# Autodesk Inventor assembly: robo-gardener-2
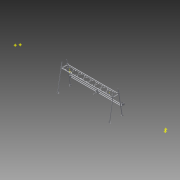
[picture p0: Inventor's stored thumbnail of the model, 180x180]
Saved by Autodesk Inventor 2013 (Build 170138000, 138)
## iProperties
Created: 2013-09-24
Part Number: robo-gardener-2
Document SubType Name: Assembly
Designer: Admin
Author: Admin
## Documents named in this file (12)
- Z:\Dropbox\projects\robo-gardener\robo-gardener-2.iam
- Z:\Dropbox\projects\robo-gardener\3d-parts\light-mount.ipt
- Z:\Dropbox\projects\robo-gardener\3d-parts\rod-long.ipt
- Z:\Dropbox\projects\robo-gardener\3d-parts\carriage-back.ipt
- Z:\Dropbox\projects\robo-gardener\3d-parts\carriage-front.ipt
- Z:\Dropbox\projects\robo-gardener\robo-gardener-2\Design Accelerator\Synchronous Belts Transmission1.iam
- Z:\Dropbox\projects\robo-gardener\3d-parts\belt-clamp.ipt
- Z:\Dropbox\projects\robo-gardener\3d-parts\motor-mount.ipt
- Z:\Dropbox\projects\robo-gardener\3d-parts\idler-mount.ipt
- Z:\Dropbox\projects\robo-gardener\3d-parts\top-connector.ipt
- Z:\Dropbox\projects\robo-gardener\3d-parts\rod-short.ipt
- Z:\Dropbox\projects\robo-gardener\3d-parts\foot.ipt
## Components (28 placed, 11 different names)
1. rod-long:1 — Insert:1, Flush:7, Insert:9, Insert:11
2. rod-long:2 — Insert:2, Mate:13, Insert:8, Insert:10
3. carriage-back:1 — Mate:1, Mate:2, Flush:9, Flush:10, Angle:1, Mate:12, Flush:13
4. carriage-front:1 — Flush:6, Mate:3, Flush:9, Flush:10, Mate:4, Flush:12, Insert:3, Insert:4, Mate:7
5. rod-long:3 — Flush:7, Flush:8, Mate:1, Mate:3, Flush:11, Mate:14, Insert:7
6. rod-long:4 — Flush:8, Mate:2, Mate:15, Insert:5, Insert:6
7. Synchronous Belts Transmission:1 [sub-assembly] — Mate:4, Mate:6, Mate:7
8. belt-clamp:1 — Flush:12, Insert:3, Insert:4
9. motor-mount:1 — Insert:5, Angle:3
10. idler-mount:1 — Insert:6, Insert:7
11. top-connector:1 — Insert:8, Insert:9, Mate:23, Mate:24
12. top-connector:2 — Insert:10, Insert:11, Mate:25, Mate:26
13. rod-short:1 — Mate:23, Insert:16
14. rod-short:2 — Mate:25, Insert:12
15. rod-short:3 — Mate:26, Insert:18
16. rod-short:4 — Mate:24, Insert:17
17. foot:1 — Insert:12, Flush:15, Flush:16, Flush:17
18. foot:2 — Insert:18, Flush:16
19. foot:3 — Insert:17, Flush:15
20. foot:4 — Insert:16, Flush:17
21. light-mount:1 — Insert:1, Insert:2, Mate:8, Flush:13
22. light-mount:2
23. light-mount:3
24. light-mount:4
25. light-mount:5
26. light-mount:6
27. light-mount:7
28. light-mount:8 — Angle:1, Mate:9
## Component patterns: (8 elements, first: light-mount:1)
## Relationships (55: Mate 25, Insert 15, Flush 12, Angle 3)
- Insert:1 (-30 mm): rod-long:1 ↔ light-mount:1
- Insert:2 (-30 mm): rod-long:2 ↔ light-mount:1
- Flush:6 (3.048 mm): carriage-front:1
- Flush:7: rod-long:1 ↔ rod-long:3
- Flush:8: rod-long:3 ↔ rod-long:4
- Mate:1: carriage-back:1 ↔ rod-long:3
- Mate:2: carriage-back:1 ↔ rod-long:4
- Mate:3: carriage-front:1 ↔ rod-long:3
- Flush:9: carriage-back:1 ↔ carriage-front:1
- Flush:10: carriage-back:1 ↔ carriage-front:1
- Angle:1 (0 deg): carriage-back:1 ↔ light-mount:8
- Mate:4 (8.25 mm): carriage-front:1 ↔ Synchronous Belts Transmission:1
- Flush:11 (35.56 mm): rod-long:3
- Mate:6: Synchronous Belts Transmission:1
- Flush:12: carriage-front:1 ↔ belt-clamp:1
- Insert:3: carriage-front:1 ↔ belt-clamp:1
- Insert:4: carriage-front:1 ↔ belt-clamp:1
- Mate:7: carriage-front:1 ↔ Synchronous Belts Transmission:1
- Mate:8: light-mount:1
- Mate:9: light-mount:8
- Mate:10
- Mate:11
- Mate:12 (30 mm): carriage-back:1
- Flush:13 (200 mm): carriage-back:1 ↔ light-mount:1
- Mate:13: rod-long:2
- Mate:14: rod-long:3
- Mate:15: rod-long:4
- Mate:16
- Mate:17
- Flush:14 (20 mm)
- Mate:18
- Angle:2 (90 deg)
- Mate:19
- Mate:20
- Mate:21
- Mate:22
- Insert:5 (-20 mm): rod-long:4 ↔ motor-mount:1
- Angle:3 (0 deg): motor-mount:1
- Insert:6: rod-long:4 ↔ idler-mount:1
- Insert:7: rod-long:3 ↔ idler-mount:1
- Insert:8: rod-long:2 ↔ top-connector:1
- Insert:9: rod-long:1 ↔ top-connector:1
- Insert:10: rod-long:2 ↔ top-connector:2
- Insert:11: rod-long:1 ↔ top-connector:2
- Mate:23: top-connector:1 ↔ rod-short:1
- Mate:24: top-connector:1 ↔ rod-short:4
- Mate:25: top-connector:2 ↔ rod-short:2
- Mate:26: top-connector:2 ↔ rod-short:3
- Insert:12: rod-short:2 ↔ foot:1
- Insert:16: rod-short:1 ↔ foot:4
- Insert:17: rod-short:4 ↔ foot:3
- Insert:18: rod-short:3 ↔ foot:2
- Flush:15: foot:1 ↔ foot:3
- Flush:16: foot:1 ↔ foot:2
- Flush:17: foot:1 ↔ foot:4
